# Autodesk Inventor assembly: narrow high rectangular -0
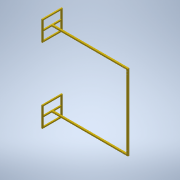
[picture p0: Inventor's stored thumbnail of the model, 180x180]
Saved by Autodesk Inventor 2021 (Build 250183000, 183)
## iProperties
Created: 2024-04-18
Part Number: narrow high rectangular -0
Document SubType Name: Assembly
Designer: Michal
Author: Michal
## Documents named in this file (7)
- C:\Users\Michal\Documents\GitHub\PNW_PhotoBoothFrame_3D\narrow high rectangular\narrow high rectangular -0.iam
- C:\Users\Michal\Documents\GitHub\PNW_PhotoBoothFrame_3D\narrow high rectangular\narrow high rectangular -0.1.iam
- C:\Users\Michal\Documents\GitHub\PNW_PhotoBoothFrame_3D\narrow high rectangular\narrow high rectangular -0.2.iam
- C:\Users\Michal\Documents\GitHub\PNW_PhotoBoothFrame_3D\narrow high rectangular\beam 30x30x2 -1.ipt
- C:\Users\Michal\Documents\GitHub\PNW_PhotoBoothFrame_3D\M8x15.ipt
- C:\Users\Michal\Documents\GitHub\PNW_PhotoBoothFrame_3D\narrow high rectangular\beam 30x30x2 -2.ipt
- C:\Users\Michal\Documents\GitHub\PNW_PhotoBoothFrame_3D\narrow high rectangular\beam 30x30x2 -3.ipt
## Components (19 placed, 6 different names)
1. narrow high rectangular -0.1:1 [sub-assembly] — Flush:1, Flush:2, Mate:1, Flush:3, Mate:2, Mate:3, Mate:5
2. narrow high rectangular -0.1:2 [sub-assembly] — Flush:1, Flush:2, Mate:10, Flush:4, Flush:5, Mate:11, Mate:18, Mate:20
3. narrow high rectangular -0.2:1 [sub-assembly] — Mate:12, Mate:13, Mate:14, Mate:15, Mate:22, Mate:24, Mate:26, Mate:28
4. narrow high rectangular -0.2:2 [sub-assembly] — Mate:7, Mate:8, Mate:9, Mate:17, Mate:30, Mate:32, Mate:34, Mate:36
5. beam 30x30x2 -1:1 — Mate:1, Flush:3, Mate:2, Mate:4, Mate:6, Mate:7, Mate:8, Mate:9, Mate:31, Mate:33
6. M8x15:1 — Mate:3, Mate:4
7. M8x15:2 — Mate:5, Mate:6
8. beam 30x30x2 -2:1 — Mate:10, Flush:4, Flush:5, Mate:11, Mate:12, Mate:13, Mate:14, Flush:6, Mate:19, Mate:21, Mate:23, Mate:25
9. beam 30x30x2 -3:1 — Flush:6, Mate:15, Mate:17, Mate:27, Mate:29, Mate:35, Mate:37
10. M8x15:3 — Mate:18, Mate:19
11. M8x15:4 — Mate:20, Mate:21
12. M8x15:5 — Mate:22, Mate:23
13. M8x15:6 — Mate:24, Mate:25
14. M8x15:7 — Mate:26, Mate:27
15. M8x15:8 — Mate:28, Mate:29
16. M8x15:9 — Mate:30, Mate:31
17. M8x15:10 — Mate:32, Mate:33
18. M8x15:11 — Mate:34, Mate:35
19. M8x15:12 — Mate:36, Mate:37
## Relationships (42: Mate 36, Flush 6)
- Flush:1: narrow high rectangular -0.1:1 ↔ narrow high rectangular -0.1:2
- Flush:2: narrow high rectangular -0.1:1 ↔ narrow high rectangular -0.1:2
- Mate:1: narrow high rectangular -0.1:1 ↔ beam 30x30x2 -1:1
- Flush:3: narrow high rectangular -0.1:1 ↔ beam 30x30x2 -1:1
- Mate:2: narrow high rectangular -0.1:1 ↔ beam 30x30x2 -1:1
- Mate:3: narrow high rectangular -0.1:1 ↔ M8x15:1
- Mate:4: beam 30x30x2 -1:1 ↔ M8x15:1
- Mate:5: narrow high rectangular -0.1:1 ↔ M8x15:2
- Mate:6: beam 30x30x2 -1:1 ↔ M8x15:2
- Mate:7: narrow high rectangular -0.2:2 ↔ beam 30x30x2 -1:1
- Mate:8: narrow high rectangular -0.2:2 ↔ beam 30x30x2 -1:1
- Mate:9: narrow high rectangular -0.2:2 ↔ beam 30x30x2 -1:1
- Mate:10: narrow high rectangular -0.1:2 ↔ beam 30x30x2 -2:1
- Flush:4: narrow high rectangular -0.1:2 ↔ beam 30x30x2 -2:1
- Flush:5: narrow high rectangular -0.1:2 ↔ beam 30x30x2 -2:1
- Mate:11: narrow high rectangular -0.1:2 ↔ beam 30x30x2 -2:1
- Mate:12: narrow high rectangular -0.2:1 ↔ beam 30x30x2 -2:1
- Mate:13: narrow high rectangular -0.2:1 ↔ beam 30x30x2 -2:1
- Mate:14: narrow high rectangular -0.2:1 ↔ beam 30x30x2 -2:1
- Flush:6: beam 30x30x2 -2:1 ↔ beam 30x30x2 -3:1
- Mate:15: narrow high rectangular -0.2:1 ↔ beam 30x30x2 -3:1
- Mate:17: narrow high rectangular -0.2:2 ↔ beam 30x30x2 -3:1
- Mate:18: narrow high rectangular -0.1:2 ↔ M8x15:3
- Mate:19: beam 30x30x2 -2:1 ↔ M8x15:3
- Mate:20: narrow high rectangular -0.1:2 ↔ M8x15:4
- Mate:21: beam 30x30x2 -2:1 ↔ M8x15:4
- Mate:22: narrow high rectangular -0.2:1 ↔ M8x15:5
- Mate:23: beam 30x30x2 -2:1 ↔ M8x15:5
- Mate:24: narrow high rectangular -0.2:1 ↔ M8x15:6
- Mate:25: beam 30x30x2 -2:1 ↔ M8x15:6
- Mate:26: narrow high rectangular -0.2:1 ↔ M8x15:7
- Mate:27: beam 30x30x2 -3:1 ↔ M8x15:7
- Mate:28: narrow high rectangular -0.2:1 ↔ M8x15:8
- Mate:29: beam 30x30x2 -3:1 ↔ M8x15:8
- Mate:30: narrow high rectangular -0.2:2 ↔ M8x15:9
- Mate:31: beam 30x30x2 -1:1 ↔ M8x15:9
- Mate:32: narrow high rectangular -0.2:2 ↔ M8x15:10
- Mate:33: beam 30x30x2 -1:1 ↔ M8x15:10
- Mate:34: narrow high rectangular -0.2:2 ↔ M8x15:11
- Mate:35: beam 30x30x2 -3:1 ↔ M8x15:11
- Mate:36: narrow high rectangular -0.2:2 ↔ M8x15:12
- Mate:37: beam 30x30x2 -3:1 ↔ M8x15:12
